(part 1 of 2)
# Autodesk Inventor assembly: eMachineShop.20
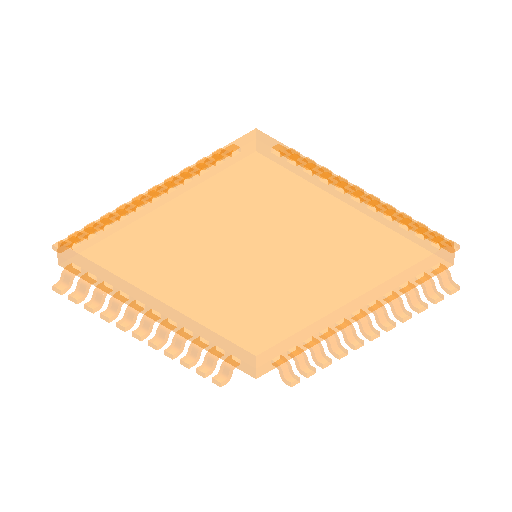
[picture p0: Inventor's stored thumbnail of the model, 512x512]
Saved by Autodesk Inventor 2026.1 (Build 301233000, 233)
## iProperties
Created: 2025-10-01
Part Number: eMachineShop.20
Document SubType Name: Assembly
Designer: gianm
Author: gianm
## Documents named in this file (583)
- D:\Tesis\Modelo 3D\CAD\Electronicos\MC15A_V5\MC15A_V5_1779569544.214\MC15A_V5_1779569544.214\eMachineShop.20.iam
- D:\Tesis\Modelo 3D\CAD\Electronicos\MC15A_V5\MC15A_V5_1779569544.214\MC15A_V5_1779569544.214\eMachineShop.20.1.ipt
- D:\Tesis\Modelo 3D\CAD\Electronicos\MC15A_V5\MC15A_V5_1779569544.214\MC15A_V5_1779569544.214\eMachineShop.20.2.ipt
- D:\Tesis\Modelo 3D\CAD\Electronicos\MC15A_V5\MC15A_V5_1779569544.214\MC15A_V5_1779569544.214\eMachineShop.20.3.ipt
- D:\Tesis\Modelo 3D\CAD\Electronicos\MC15A_V5\MC15A_V5_1779569544.214\MC15A_V5_1779569544.214\eMachineShop.20.4.ipt
- D:\Tesis\Modelo 3D\CAD\Electronicos\MC15A_V5\MC15A_V5_1779569544.214\MC15A_V5_1779569544.214\eMachineShop.20.5.ipt
- D:\Tesis\Modelo 3D\CAD\Electronicos\MC15A_V5\MC15A_V5_1779569544.214\MC15A_V5_1779569544.214\eMachineShop.20.6.ipt
- D:\Tesis\Modelo 3D\CAD\Electronicos\MC15A_V5\MC15A_V5_1779569544.214\MC15A_V5_1779569544.214\eMachineShop.20.7.ipt
- D:\Tesis\Modelo 3D\CAD\Electronicos\MC15A_V5\MC15A_V5_1779569544.214\MC15A_V5_1779569544.214\eMachineShop.20.8.ipt
- D:\Tesis\Modelo 3D\CAD\Electronicos\MC15A_V5\MC15A_V5_1779569544.214\MC15A_V5_1779569544.214\eMachineShop.20.9.ipt
- D:\Tesis\Modelo 3D\CAD\Electronicos\MC15A_V5\MC15A_V5_1779569544.214\MC15A_V5_1779569544.214\eMachineShop.20.10.ipt
- D:\Tesis\Modelo 3D\CAD\Electronicos\MC15A_V5\MC15A_V5_1779569544.214\MC15A_V5_1779569544.214\eMachineShop.20.11.ipt
- D:\Tesis\Modelo 3D\CAD\Electronicos\MC15A_V5\MC15A_V5_1779569544.214\MC15A_V5_1779569544.214\eMachineShop.20.12.ipt
- D:\Tesis\Modelo 3D\CAD\Electronicos\MC15A_V5\MC15A_V5_1779569544.214\MC15A_V5_1779569544.214\eMachineShop.20.13.ipt
- D:\Tesis\Modelo 3D\CAD\Electronicos\MC15A_V5\MC15A_V5_1779569544.214\MC15A_V5_1779569544.214\eMachineShop.20.14.ipt
- D:\Tesis\Modelo 3D\CAD\Electronicos\MC15A_V5\MC15A_V5_1779569544.214\MC15A_V5_1779569544.214\eMachineShop.20.15.ipt
- D:\Tesis\Modelo 3D\CAD\Electronicos\MC15A_V5\MC15A_V5_1779569544.214\MC15A_V5_1779569544.214\eMachineShop.20.16.ipt
- D:\Tesis\Modelo 3D\CAD\Electronicos\MC15A_V5\MC15A_V5_1779569544.214\MC15A_V5_1779569544.214\eMachineShop.20.17.ipt
- D:\Tesis\Modelo 3D\CAD\Electronicos\MC15A_V5\MC15A_V5_1779569544.214\MC15A_V5_1779569544.214\eMachineShop.20.18.ipt
- D:\Tesis\Modelo 3D\CAD\Electronicos\MC15A_V5\MC15A_V5_1779569544.214\MC15A_V5_1779569544.214\eMachineShop.20.19.ipt
- D:\Tesis\Modelo 3D\CAD\Electronicos\MC15A_V5\MC15A_V5_1779569544.214\MC15A_V5_1779569544.214\eMachineShop.20.20.ipt
- D:\Tesis\Modelo 3D\CAD\Electronicos\MC15A_V5\MC15A_V5_1779569544.214\MC15A_V5_1779569544.214\eMachineShop.20.21.ipt
- D:\Tesis\Modelo 3D\CAD\Electronicos\MC15A_V5\MC15A_V5_1779569544.214\MC15A_V5_1779569544.214\eMachineShop.20.22.ipt
- D:\Tesis\Modelo 3D\CAD\Electronicos\MC15A_V5\MC15A_V5_1779569544.214\MC15A_V5_1779569544.214\eMachineShop.20.23.ipt
- D:\Tesis\Modelo 3D\CAD\Electronicos\MC15A_V5\MC15A_V5_1779569544.214\MC15A_V5_1779569544.214\eMachineShop.20.24.ipt
- D:\Tesis\Modelo 3D\CAD\Electronicos\MC15A_V5\MC15A_V5_1779569544.214\MC15A_V5_1779569544.214\eMachineShop.20.25.ipt
- D:\Tesis\Modelo 3D\CAD\Electronicos\MC15A_V5\MC15A_V5_1779569544.214\MC15A_V5_1779569544.214\eMachineShop.20.26.ipt
- D:\Tesis\Modelo 3D\CAD\Electronicos\MC15A_V5\MC15A_V5_1779569544.214\MC15A_V5_1779569544.214\eMachineShop.20.27.ipt
- D:\Tesis\Modelo 3D\CAD\Electronicos\MC15A_V5\MC15A_V5_1779569544.214\MC15A_V5_1779569544.214\eMachineShop.20.28.ipt
- D:\Tesis\Modelo 3D\CAD\Electronicos\MC15A_V5\MC15A_V5_1779569544.214\MC15A_V5_1779569544.214\eMachineShop.20.29.ipt
- D:\Tesis\Modelo 3D\CAD\Electronicos\MC15A_V5\MC15A_V5_1779569544.214\MC15A_V5_1779569544.214\eMachineShop.20.30.ipt
- D:\Tesis\Modelo 3D\CAD\Electronicos\MC15A_V5\MC15A_V5_1779569544.214\MC15A_V5_1779569544.214\eMachineShop.20.31.ipt
- D:\Tesis\Modelo 3D\CAD\Electronicos\MC15A_V5\MC15A_V5_1779569544.214\MC15A_V5_1779569544.214\eMachineShop.20.32.ipt
- D:\Tesis\Modelo 3D\CAD\Electronicos\MC15A_V5\MC15A_V5_1779569544.214\MC15A_V5_1779569544.214\eMachineShop.20.33.ipt
- D:\Tesis\Modelo 3D\CAD\Electronicos\MC15A_V5\MC15A_V5_1779569544.214\MC15A_V5_1779569544.214\eMachineShop.20.34.ipt
- D:\Tesis\Modelo 3D\CAD\Electronicos\MC15A_V5\MC15A_V5_1779569544.214\MC15A_V5_1779569544.214\eMachineShop.20.35.ipt
- D:\Tesis\Modelo 3D\CAD\Electronicos\MC15A_V5\MC15A_V5_1779569544.214\MC15A_V5_1779569544.214\eMachineShop.20.36.ipt
- D:\Tesis\Modelo 3D\CAD\Electronicos\MC15A_V5\MC15A_V5_1779569544.214\MC15A_V5_1779569544.214\eMachineShop.20.37.ipt
- D:\Tesis\Modelo 3D\CAD\Electronicos\MC15A_V5\MC15A_V5_1779569544.214\MC15A_V5_1779569544.214\eMachineShop.20.38.ipt
- D:\Tesis\Modelo 3D\CAD\Electronicos\MC15A_V5\MC15A_V5_1779569544.214\MC15A_V5_1779569544.214\eMachineShop.20.39.ipt
- D:\Tesis\Modelo 3D\CAD\Electronicos\MC15A_V5\MC15A_V5_1779569544.214\MC15A_V5_1779569544.214\eMachineShop.20.40.ipt
- D:\Tesis\Modelo 3D\CAD\Electronicos\MC15A_V5\MC15A_V5_1779569544.214\MC15A_V5_1779569544.214\eMachineShop.20.41.ipt
- D:\Tesis\Modelo 3D\CAD\Electronicos\MC15A_V5\MC15A_V5_1779569544.214\MC15A_V5_1779569544.214\eMachineShop.20.42.ipt
- D:\Tesis\Modelo 3D\CAD\Electronicos\MC15A_V5\MC15A_V5_1779569544.214\MC15A_V5_1779569544.214\eMachineShop.20.43.ipt
- D:\Tesis\Modelo 3D\CAD\Electronicos\MC15A_V5\MC15A_V5_1779569544.214\MC15A_V5_1779569544.214\eMachineShop.20.44.ipt
- D:\Tesis\Modelo 3D\CAD\Electronicos\MC15A_V5\MC15A_V5_1779569544.214\MC15A_V5_1779569544.214\eMachineShop.20.45.ipt
- D:\Tesis\Modelo 3D\CAD\Electronicos\MC15A_V5\MC15A_V5_1779569544.214\MC15A_V5_1779569544.214\eMachineShop.20.46.ipt
- D:\Tesis\Modelo 3D\CAD\Electronicos\MC15A_V5\MC15A_V5_1779569544.214\MC15A_V5_1779569544.214\eMachineShop.20.47.ipt
- D:\Tesis\Modelo 3D\CAD\Electronicos\MC15A_V5\MC15A_V5_1779569544.214\MC15A_V5_1779569544.214\eMachineShop.20.48.ipt
- D:\Tesis\Modelo 3D\CAD\Electronicos\MC15A_V5\MC15A_V5_1779569544.214\MC15A_V5_1779569544.214\eMachineShop.20.49.ipt
- D:\Tesis\Modelo 3D\CAD\Electronicos\MC15A_V5\MC15A_V5_1779569544.214\MC15A_V5_1779569544.214\eMachineShop.20.50.ipt
- D:\Tesis\Modelo 3D\CAD\Electronicos\MC15A_V5\MC15A_V5_1779569544.214\MC15A_V5_1779569544.214\eMachineShop.20.51.ipt
- D:\Tesis\Modelo 3D\CAD\Electronicos\MC15A_V5\MC15A_V5_1779569544.214\MC15A_V5_1779569544.214\eMachineShop.20.52.ipt
- D:\Tesis\Modelo 3D\CAD\Electronicos\MC15A_V5\MC15A_V5_1779569544.214\MC15A_V5_1779569544.214\eMachineShop.20.53.ipt
- D:\Tesis\Modelo 3D\CAD\Electronicos\MC15A_V5\MC15A_V5_1779569544.214\MC15A_V5_1779569544.214\eMachineShop.20.54.ipt
- D:\Tesis\Modelo 3D\CAD\Electronicos\MC15A_V5\MC15A_V5_1779569544.214\MC15A_V5_1779569544.214\eMachineShop.20.55.ipt
- D:\Tesis\Modelo 3D\CAD\Electronicos\MC15A_V5\MC15A_V5_1779569544.214\MC15A_V5_1779569544.214\eMachineShop.20.56.ipt
- D:\Tesis\Modelo 3D\CAD\Electronicos\MC15A_V5\MC15A_V5_1779569544.214\MC15A_V5_1779569544.214\eMachineShop.20.57.ipt
- D:\Tesis\Modelo 3D\CAD\Electronicos\MC15A_V5\MC15A_V5_1779569544.214\MC15A_V5_1779569544.214\eMachineShop.20.58.ipt
- D:\Tesis\Modelo 3D\CAD\Electronicos\MC15A_V5\MC15A_V5_1779569544.214\MC15A_V5_1779569544.214\eMachineShop.20.59.ipt
- D:\Tesis\Modelo 3D\CAD\Electronicos\MC15A_V5\MC15A_V5_1779569544.214\MC15A_V5_1779569544.214\eMachineShop.20.60.ipt
- D:\Tesis\Modelo 3D\CAD\Electronicos\MC15A_V5\MC15A_V5_1779569544.214\MC15A_V5_1779569544.214\eMachineShop.20.61.ipt
- D:\Tesis\Modelo 3D\CAD\Electronicos\MC15A_V5\MC15A_V5_1779569544.214\MC15A_V5_1779569544.214\eMachineShop.20.62.ipt
- D:\Tesis\Modelo 3D\CAD\Electronicos\MC15A_V5\MC15A_V5_1779569544.214\MC15A_V5_1779569544.214\eMachineShop.20.63.ipt
- D:\Tesis\Modelo 3D\CAD\Electronicos\MC15A_V5\MC15A_V5_1779569544.214\MC15A_V5_1779569544.214\eMachineShop.20.64.ipt
- D:\Tesis\Modelo 3D\CAD\Electronicos\MC15A_V5\MC15A_V5_1779569544.214\MC15A_V5_1779569544.214\eMachineShop.20.65.ipt
- D:\Tesis\Modelo 3D\CAD\Electronicos\MC15A_V5\MC15A_V5_1779569544.214\MC15A_V5_1779569544.214\eMachineShop.20.66.ipt
- D:\Tesis\Modelo 3D\CAD\Electronicos\MC15A_V5\MC15A_V5_1779569544.214\MC15A_V5_1779569544.214\eMachineShop.20.67.ipt
- D:\Tesis\Modelo 3D\CAD\Electronicos\MC15A_V5\MC15A_V5_1779569544.214\MC15A_V5_1779569544.214\eMachineShop.20.68.ipt
- D:\Tesis\Modelo 3D\CAD\Electronicos\MC15A_V5\MC15A_V5_1779569544.214\MC15A_V5_1779569544.214\eMachineShop.20.69.ipt
- D:\Tesis\Modelo 3D\CAD\Electronicos\MC15A_V5\MC15A_V5_1779569544.214\MC15A_V5_1779569544.214\eMachineShop.20.70.ipt
- D:\Tesis\Modelo 3D\CAD\Electronicos\MC15A_V5\MC15A_V5_1779569544.214\MC15A_V5_1779569544.214\eMachineShop.20.71.ipt
- D:\Tesis\Modelo 3D\CAD\Electronicos\MC15A_V5\MC15A_V5_1779569544.214\MC15A_V5_1779569544.214\eMachineShop.20.72.ipt
- D:\Tesis\Modelo 3D\CAD\Electronicos\MC15A_V5\MC15A_V5_1779569544.214\MC15A_V5_1779569544.214\eMachineShop.20.73.ipt
- D:\Tesis\Modelo 3D\CAD\Electronicos\MC15A_V5\MC15A_V5_1779569544.214\MC15A_V5_1779569544.214\eMachineShop.20.74.ipt
- D:\Tesis\Modelo 3D\CAD\Electronicos\MC15A_V5\MC15A_V5_1779569544.214\MC15A_V5_1779569544.214\eMachineShop.20.75.ipt
- D:\Tesis\Modelo 3D\CAD\Electronicos\MC15A_V5\MC15A_V5_1779569544.214\MC15A_V5_1779569544.214\eMachineShop.20.76.ipt
- D:\Tesis\Modelo 3D\CAD\Electronicos\MC15A_V5\MC15A_V5_1779569544.214\MC15A_V5_1779569544.214\eMachineShop.20.77.ipt
- D:\Tesis\Modelo 3D\CAD\Electronicos\MC15A_V5\MC15A_V5_1779569544.214\MC15A_V5_1779569544.214\eMachineShop.20.78.ipt
- D:\Tesis\Modelo 3D\CAD\Electronicos\MC15A_V5\MC15A_V5_1779569544.214\MC15A_V5_1779569544.214\eMachineShop.20.79.ipt
- D:\Tesis\Modelo 3D\CAD\Electronicos\MC15A_V5\MC15A_V5_1779569544.214\MC15A_V5_1779569544.214\eMachineShop.20.80.ipt
- D:\Tesis\Modelo 3D\CAD\Electronicos\MC15A_V5\MC15A_V5_1779569544.214\MC15A_V5_1779569544.214\eMachineShop.20.81.ipt
- D:\Tesis\Modelo 3D\CAD\Electronicos\MC15A_V5\MC15A_V5_1779569544.214\MC15A_V5_1779569544.214\eMachineShop.20.82.ipt
- D:\Tesis\Modelo 3D\CAD\Electronicos\MC15A_V5\MC15A_V5_1779569544.214\MC15A_V5_1779569544.214\eMachineShop.20.83.ipt
- D:\Tesis\Modelo 3D\CAD\Electronicos\MC15A_V5\MC15A_V5_1779569544.214\MC15A_V5_1779569544.214\eMachineShop.20.84.ipt
- D:\Tesis\Modelo 3D\CAD\Electronicos\MC15A_V5\MC15A_V5_1779569544.214\MC15A_V5_1779569544.214\eMachineShop.20.85.ipt
- D:\Tesis\Modelo 3D\CAD\Electronicos\MC15A_V5\MC15A_V5_1779569544.214\MC15A_V5_1779569544.214\eMachineShop.20.86.ipt
- D:\Tesis\Modelo 3D\CAD\Electronicos\MC15A_V5\MC15A_V5_1779569544.214\MC15A_V5_1779569544.214\eMachineShop.20.87.ipt
- D:\Tesis\Modelo 3D\CAD\Electronicos\MC15A_V5\MC15A_V5_1779569544.214\MC15A_V5_1779569544.214\eMachineShop.20.88.ipt
- D:\Tesis\Modelo 3D\CAD\Electronicos\MC15A_V5\MC15A_V5_1779569544.214\MC15A_V5_1779569544.214\eMachineShop.20.89.ipt
- D:\Tesis\Modelo 3D\CAD\Electronicos\MC15A_V5\MC15A_V5_1779569544.214\MC15A_V5_1779569544.214\eMachineShop.20.90.ipt
- D:\Tesis\Modelo 3D\CAD\Electronicos\MC15A_V5\MC15A_V5_1779569544.214\MC15A_V5_1779569544.214\eMachineShop.20.91.ipt
- D:\Tesis\Modelo 3D\CAD\Electronicos\MC15A_V5\MC15A_V5_1779569544.214\MC15A_V5_1779569544.214\eMachineShop.20.92.ipt
- D:\Tesis\Modelo 3D\CAD\Electronicos\MC15A_V5\MC15A_V5_1779569544.214\MC15A_V5_1779569544.214\eMachineShop.20.93.ipt
- D:\Tesis\Modelo 3D\CAD\Electronicos\MC15A_V5\MC15A_V5_1779569544.214\MC15A_V5_1779569544.214\eMachineShop.20.94.ipt
- D:\Tesis\Modelo 3D\CAD\Electronicos\MC15A_V5\MC15A_V5_1779569544.214\MC15A_V5_1779569544.214\eMachineShop.20.95.ipt
- D:\Tesis\Modelo 3D\CAD\Electronicos\MC15A_V5\MC15A_V5_1779569544.214\MC15A_V5_1779569544.214\eMachineShop.20.96.ipt
- D:\Tesis\Modelo 3D\CAD\Electronicos\MC15A_V5\MC15A_V5_1779569544.214\MC15A_V5_1779569544.214\eMachineShop.20.97.ipt
- D:\Tesis\Modelo 3D\CAD\Electronicos\MC15A_V5\MC15A_V5_1779569544.214\MC15A_V5_1779569544.214\eMachineShop.20.98.ipt
- D:\Tesis\Modelo 3D\CAD\Electronicos\MC15A_V5\MC15A_V5_1779569544.214\MC15A_V5_1779569544.214\eMachineShop.20.99.ipt
- D:\Tesis\Modelo 3D\CAD\Electronicos\MC15A_V5\MC15A_V5_1779569544.214\MC15A_V5_1779569544.214\eMachineShop.20.100.ipt
- D:\Tesis\Modelo 3D\CAD\Electronicos\MC15A_V5\MC15A_V5_1779569544.214\MC15A_V5_1779569544.214\eMachineShop.20.101.ipt
- D:\Tesis\Modelo 3D\CAD\Electronicos\MC15A_V5\MC15A_V5_1779569544.214\MC15A_V5_1779569544.214\eMachineShop.20.102.ipt
- D:\Tesis\Modelo 3D\CAD\Electronicos\MC15A_V5\MC15A_V5_1779569544.214\MC15A_V5_1779569544.214\eMachineShop.20.103.ipt
- D:\Tesis\Modelo 3D\CAD\Electronicos\MC15A_V5\MC15A_V5_1779569544.214\MC15A_V5_1779569544.214\eMachineShop.20.104.ipt
- D:\Tesis\Modelo 3D\CAD\Electronicos\MC15A_V5\MC15A_V5_1779569544.214\MC15A_V5_1779569544.214\eMachineShop.20.105.ipt
- D:\Tesis\Modelo 3D\CAD\Electronicos\MC15A_V5\MC15A_V5_1779569544.214\MC15A_V5_1779569544.214\eMachineShop.20.106.ipt
- D:\Tesis\Modelo 3D\CAD\Electronicos\MC15A_V5\MC15A_V5_1779569544.214\MC15A_V5_1779569544.214\eMachineShop.20.107.ipt
- D:\Tesis\Modelo 3D\CAD\Electronicos\MC15A_V5\MC15A_V5_1779569544.214\MC15A_V5_1779569544.214\eMachineShop.20.108.ipt
- D:\Tesis\Modelo 3D\CAD\Electronicos\MC15A_V5\MC15A_V5_1779569544.214\MC15A_V5_1779569544.214\eMachineShop.20.109.ipt
- D:\Tesis\Modelo 3D\CAD\Electronicos\MC15A_V5\MC15A_V5_1779569544.214\MC15A_V5_1779569544.214\eMachineShop.20.110.ipt
- D:\Tesis\Modelo 3D\CAD\Electronicos\MC15A_V5\MC15A_V5_1779569544.214\MC15A_V5_1779569544.214\eMachineShop.20.111.ipt
- D:\Tesis\Modelo 3D\CAD\Electronicos\MC15A_V5\MC15A_V5_1779569544.214\MC15A_V5_1779569544.214\eMachineShop.20.112.ipt
- D:\Tesis\Modelo 3D\CAD\Electronicos\MC15A_V5\MC15A_V5_1779569544.214\MC15A_V5_1779569544.214\eMachineShop.20.113.ipt
- D:\Tesis\Modelo 3D\CAD\Electronicos\MC15A_V5\MC15A_V5_1779569544.214\MC15A_V5_1779569544.214\eMachineShop.20.114.ipt
- D:\Tesis\Modelo 3D\CAD\Electronicos\MC15A_V5\MC15A_V5_1779569544.214\MC15A_V5_1779569544.214\eMachineShop.20.115.ipt
- D:\Tesis\Modelo 3D\CAD\Electronicos\MC15A_V5\MC15A_V5_1779569544.214\MC15A_V5_1779569544.214\eMachineShop.20.116.ipt
- D:\Tesis\Modelo 3D\CAD\Electronicos\MC15A_V5\MC15A_V5_1779569544.214\MC15A_V5_1779569544.214\eMachineShop.20.117.ipt
- D:\Tesis\Modelo 3D\CAD\Electronicos\MC15A_V5\MC15A_V5_1779569544.214\MC15A_V5_1779569544.214\eMachineShop.20.118.ipt
- D:\Tesis\Modelo 3D\CAD\Electronicos\MC15A_V5\MC15A_V5_1779569544.214\MC15A_V5_1779569544.214\eMachineShop.20.119.ipt
- D:\Tesis\Modelo 3D\CAD\Electronicos\MC15A_V5\MC15A_V5_1779569544.214\MC15A_V5_1779569544.214\eMachineShop.20.120.ipt
- D:\Tesis\Modelo 3D\CAD\Electronicos\MC15A_V5\MC15A_V5_1779569544.214\MC15A_V5_1779569544.214\eMachineShop.20.121.ipt
- D:\Tesis\Modelo 3D\CAD\Electronicos\MC15A_V5\MC15A_V5_1779569544.214\MC15A_V5_1779569544.214\eMachineShop.20.122.ipt
- D:\Tesis\Modelo 3D\CAD\Electronicos\MC15A_V5\MC15A_V5_1779569544.214\MC15A_V5_1779569544.214\eMachineShop.20.123.ipt
- D:\Tesis\Modelo 3D\CAD\Electronicos\MC15A_V5\MC15A_V5_1779569544.214\MC15A_V5_1779569544.214\eMachineShop.20.124.ipt
- D:\Tesis\Modelo 3D\CAD\Electronicos\MC15A_V5\MC15A_V5_1779569544.214\MC15A_V5_1779569544.214\eMachineShop.20.125.ipt
- D:\Tesis\Modelo 3D\CAD\Electronicos\MC15A_V5\MC15A_V5_1779569544.214\MC15A_V5_1779569544.214\eMachineShop.20.126.ipt
- D:\Tesis\Modelo 3D\CAD\Electronicos\MC15A_V5\MC15A_V5_1779569544.214\MC15A_V5_1779569544.214\eMachineShop.20.127.ipt
- D:\Tesis\Modelo 3D\CAD\Electronicos\MC15A_V5\MC15A_V5_1779569544.214\MC15A_V5_1779569544.214\eMachineShop.20.128.ipt
- D:\Tesis\Modelo 3D\CAD\Electronicos\MC15A_V5\MC15A_V5_1779569544.214\MC15A_V5_1779569544.214\eMachineShop.20.129.ipt
- D:\Tesis\Modelo 3D\CAD\Electronicos\MC15A_V5\MC15A_V5_1779569544.214\MC15A_V5_1779569544.214\eMachineShop.20.130.ipt
- D:\Tesis\Modelo 3D\CAD\Electronicos\MC15A_V5\MC15A_V5_1779569544.214\MC15A_V5_1779569544.214\eMachineShop.20.131.ipt
- D:\Tesis\Modelo 3D\CAD\Electronicos\MC15A_V5\MC15A_V5_1779569544.214\MC15A_V5_1779569544.214\eMachineShop.20.132.ipt
- D:\Tesis\Modelo 3D\CAD\Electronicos\MC15A_V5\MC15A_V5_1779569544.214\MC15A_V5_1779569544.214\eMachineShop.20.133.ipt
- D:\Tesis\Modelo 3D\CAD\Electronicos\MC15A_V5\MC15A_V5_1779569544.214\MC15A_V5_1779569544.214\eMachineShop.20.134.ipt
- D:\Tesis\Modelo 3D\CAD\Electronicos\MC15A_V5\MC15A_V5_1779569544.214\MC15A_V5_1779569544.214\eMachineShop.20.135.ipt
- D:\Tesis\Modelo 3D\CAD\Electronicos\MC15A_V5\MC15A_V5_1779569544.214\MC15A_V5_1779569544.214\eMachineShop.20.136.ipt
- D:\Tesis\Modelo 3D\CAD\Electronicos\MC15A_V5\MC15A_V5_1779569544.214\MC15A_V5_1779569544.214\eMachineShop.20.137.ipt
- D:\Tesis\Modelo 3D\CAD\Electronicos\MC15A_V5\MC15A_V5_1779569544.214\MC15A_V5_1779569544.214\eMachineShop.20.138.ipt
- D:\Tesis\Modelo 3D\CAD\Electronicos\MC15A_V5\MC15A_V5_1779569544.214\MC15A_V5_1779569544.214\eMachineShop.20.139.ipt
- D:\Tesis\Modelo 3D\CAD\Electronicos\MC15A_V5\MC15A_V5_1779569544.214\MC15A_V5_1779569544.214\eMachineShop.20.140.ipt
- D:\Tesis\Modelo 3D\CAD\Electronicos\MC15A_V5\MC15A_V5_1779569544.214\MC15A_V5_1779569544.214\eMachineShop.20.141.ipt
- D:\Tesis\Modelo 3D\CAD\Electronicos\MC15A_V5\MC15A_V5_1779569544.214\MC15A_V5_1779569544.214\eMachineShop.20.142.ipt
- D:\Tesis\Modelo 3D\CAD\Electronicos\MC15A_V5\MC15A_V5_1779569544.214\MC15A_V5_1779569544.214\eMachineShop.20.143.ipt
- D:\Tesis\Modelo 3D\CAD\Electronicos\MC15A_V5\MC15A_V5_1779569544.214\MC15A_V5_1779569544.214\eMachineShop.20.144.ipt
- D:\Tesis\Modelo 3D\CAD\Electronicos\MC15A_V5\MC15A_V5_1779569544.214\MC15A_V5_1779569544.214\eMachineShop.20.145.ipt
- D:\Tesis\Modelo 3D\CAD\Electronicos\MC15A_V5\MC15A_V5_1779569544.214\MC15A_V5_1779569544.214\eMachineShop.20.146.ipt
- D:\Tesis\Modelo 3D\CAD\Electronicos\MC15A_V5\MC15A_V5_1779569544.214\MC15A_V5_1779569544.214\eMachineShop.20.147.ipt
- D:\Tesis\Modelo 3D\CAD\Electronicos\MC15A_V5\MC15A_V5_1779569544.214\MC15A_V5_1779569544.214\eMachineShop.20.148.ipt
- D:\Tesis\Modelo 3D\CAD\Electronicos\MC15A_V5\MC15A_V5_1779569544.214\MC15A_V5_1779569544.214\eMachineShop.20.149.ipt
- D:\Tesis\Modelo 3D\CAD\Electronicos\MC15A_V5\MC15A_V5_1779569544.214\MC15A_V5_1779569544.214\eMachineShop.20.150.ipt
- D:\Tesis\Modelo 3D\CAD\Electronicos\MC15A_V5\MC15A_V5_1779569544.214\MC15A_V5_1779569544.214\eMachineShop.20.151.ipt
- D:\Tesis\Modelo 3D\CAD\Electronicos\MC15A_V5\MC15A_V5_1779569544.214\MC15A_V5_1779569544.214\eMachineShop.20.152.ipt
- D:\Tesis\Modelo 3D\CAD\Electronicos\MC15A_V5\MC15A_V5_1779569544.214\MC15A_V5_1779569544.214\eMachineShop.20.153.ipt
- D:\Tesis\Modelo 3D\CAD\Electronicos\MC15A_V5\MC15A_V5_1779569544.214\MC15A_V5_1779569544.214\eMachineShop.20.154.ipt
- D:\Tesis\Modelo 3D\CAD\Electronicos\MC15A_V5\MC15A_V5_1779569544.214\MC15A_V5_1779569544.214\eMachineShop.20.155.ipt
- D:\Tesis\Modelo 3D\CAD\Electronicos\MC15A_V5\MC15A_V5_1779569544.214\MC15A_V5_1779569544.214\eMachineShop.20.156.ipt
- D:\Tesis\Modelo 3D\CAD\Electronicos\MC15A_V5\MC15A_V5_1779569544.214\MC15A_V5_1779569544.214\eMachineShop.20.157.ipt
- D:\Tesis\Modelo 3D\CAD\Electronicos\MC15A_V5\MC15A_V5_1779569544.214\MC15A_V5_1779569544.214\eMachineShop.20.158.ipt
- D:\Tesis\Modelo 3D\CAD\Electronicos\MC15A_V5\MC15A_V5_1779569544.214\MC15A_V5_1779569544.214\eMachineShop.20.159.ipt
- D:\Tesis\Modelo 3D\CAD\Electronicos\MC15A_V5\MC15A_V5_1779569544.214\MC15A_V5_1779569544.214\eMachineShop.20.160.ipt
- D:\Tesis\Modelo 3D\CAD\Electronicos\MC15A_V5\MC15A_V5_1779569544.214\MC15A_V5_1779569544.214\eMachineShop.20.161.ipt
- D:\Tesis\Modelo 3D\CAD\Electronicos\MC15A_V5\MC15A_V5_1779569544.214\MC15A_V5_1779569544.214\eMachineShop.20.162.ipt
- D:\Tesis\Modelo 3D\CAD\Electronicos\MC15A_V5\MC15A_V5_1779569544.214\MC15A_V5_1779569544.214\eMachineShop.20.163.ipt
- D:\Tesis\Modelo 3D\CAD\Electronicos\MC15A_V5\MC15A_V5_1779569544.214\MC15A_V5_1779569544.214\eMachineShop.20.164.ipt
- D:\Tesis\Modelo 3D\CAD\Electronicos\MC15A_V5\MC15A_V5_1779569544.214\MC15A_V5_1779569544.214\eMachineShop.20.165.ipt
- D:\Tesis\Modelo 3D\CAD\Electronicos\MC15A_V5\MC15A_V5_1779569544.214\MC15A_V5_1779569544.214\eMachineShop.20.166.ipt
- D:\Tesis\Modelo 3D\CAD\Electronicos\MC15A_V5\MC15A_V5_1779569544.214\MC15A_V5_1779569544.214\eMachineShop.20.167.ipt
- D:\Tesis\Modelo 3D\CAD\Electronicos\MC15A_V5\MC15A_V5_1779569544.214\MC15A_V5_1779569544.214\eMachineShop.20.168.ipt
- D:\Tesis\Modelo 3D\CAD\Electronicos\MC15A_V5\MC15A_V5_1779569544.214\MC15A_V5_1779569544.214\eMachineShop.20.169.ipt
- D:\Tesis\Modelo 3D\CAD\Electronicos\MC15A_V5\MC15A_V5_1779569544.214\MC15A_V5_1779569544.214\eMachineShop.20.170.ipt
- D:\Tesis\Modelo 3D\CAD\Electronicos\MC15A_V5\MC15A_V5_1779569544.214\MC15A_V5_1779569544.214\eMachineShop.20.171.ipt
- D:\Tesis\Modelo 3D\CAD\Electronicos\MC15A_V5\MC15A_V5_1779569544.214\MC15A_V5_1779569544.214\eMachineShop.20.172.ipt
- D:\Tesis\Modelo 3D\CAD\Electronicos\MC15A_V5\MC15A_V5_1779569544.214\MC15A_V5_1779569544.214\eMachineShop.20.173.ipt
- D:\Tesis\Modelo 3D\CAD\Electronicos\MC15A_V5\MC15A_V5_1779569544.214\MC15A_V5_1779569544.214\eMachineShop.20.174.ipt
- D:\Tesis\Modelo 3D\CAD\Electronicos\MC15A_V5\MC15A_V5_1779569544.214\MC15A_V5_1779569544.214\eMachineShop.20.175.ipt
- D:\Tesis\Modelo 3D\CAD\Electronicos\MC15A_V5\MC15A_V5_1779569544.214\MC15A_V5_1779569544.214\eMachineShop.20.176.ipt
- D:\Tesis\Modelo 3D\CAD\Electronicos\MC15A_V5\MC15A_V5_1779569544.214\MC15A_V5_1779569544.214\eMachineShop.20.177.ipt
- D:\Tesis\Modelo 3D\CAD\Electronicos\MC15A_V5\MC15A_V5_1779569544.214\MC15A_V5_1779569544.214\eMachineShop.20.178.ipt
- D:\Tesis\Modelo 3D\CAD\Electronicos\MC15A_V5\MC15A_V5_1779569544.214\MC15A_V5_1779569544.214\eMachineShop.20.179.ipt
- D:\Tesis\Modelo 3D\CAD\Electronicos\MC15A_V5\MC15A_V5_1779569544.214\MC15A_V5_1779569544.214\eMachineShop.20.180.ipt
- D:\Tesis\Modelo 3D\CAD\Electronicos\MC15A_V5\MC15A_V5_1779569544.214\MC15A_V5_1779569544.214\eMachineShop.20.181.ipt
- D:\Tesis\Modelo 3D\CAD\Electronicos\MC15A_V5\MC15A_V5_1779569544.214\MC15A_V5_1779569544.214\eMachineShop.20.182.ipt
- D:\Tesis\Modelo 3D\CAD\Electronicos\MC15A_V5\MC15A_V5_1779569544.214\MC15A_V5_1779569544.214\eMachineShop.20.183.ipt
- D:\Tesis\Modelo 3D\CAD\Electronicos\MC15A_V5\MC15A_V5_1779569544.214\MC15A_V5_1779569544.214\eMachineShop.20.184.ipt
- D:\Tesis\Modelo 3D\CAD\Electronicos\MC15A_V5\MC15A_V5_1779569544.214\MC15A_V5_1779569544.214\eMachineShop.20.185.ipt
- D:\Tesis\Modelo 3D\CAD\Electronicos\MC15A_V5\MC15A_V5_1779569544.214\MC15A_V5_1779569544.214\eMachineShop.20.186.ipt
- D:\Tesis\Modelo 3D\CAD\Electronicos\MC15A_V5\MC15A_V5_1779569544.214\MC15A_V5_1779569544.214\eMachineShop.20.187.ipt
- D:\Tesis\Modelo 3D\CAD\Electronicos\MC15A_V5\MC15A_V5_1779569544.214\MC15A_V5_1779569544.214\eMachineShop.20.188.ipt
- D:\Tesis\Modelo 3D\CAD\Electronicos\MC15A_V5\MC15A_V5_1779569544.214\MC15A_V5_1779569544.214\eMachineShop.20.189.ipt
- D:\Tesis\Modelo 3D\CAD\Electronicos\MC15A_V5\MC15A_V5_1779569544.214\MC15A_V5_1779569544.214\eMachineShop.20.190.ipt
- D:\Tesis\Modelo 3D\CAD\Electronicos\MC15A_V5\MC15A_V5_1779569544.214\MC15A_V5_1779569544.214\eMachineShop.20.191.ipt
- D:\Tesis\Modelo 3D\CAD\Electronicos\MC15A_V5\MC15A_V5_1779569544.214\MC15A_V5_1779569544.214\eMachineShop.20.192.ipt
- D:\Tesis\Modelo 3D\CAD\Electronicos\MC15A_V5\MC15A_V5_1779569544.214\MC15A_V5_1779569544.214\eMachineShop.20.193.ipt
- D:\Tesis\Modelo 3D\CAD\Electronicos\MC15A_V5\MC15A_V5_1779569544.214\MC15A_V5_1779569544.214\eMachineShop.20.194.ipt
- D:\Tesis\Modelo 3D\CAD\Electronicos\MC15A_V5\MC15A_V5_1779569544.214\MC15A_V5_1779569544.214\eMachineShop.20.195.ipt
- D:\Tesis\Modelo 3D\CAD\Electronicos\MC15A_V5\MC15A_V5_1779569544.214\MC15A_V5_1779569544.214\eMachineShop.20.196.ipt
- D:\Tesis\Modelo 3D\CAD\Electronicos\MC15A_V5\MC15A_V5_1779569544.214\MC15A_V5_1779569544.214\eMachineShop.20.197.ipt
- D:\Tesis\Modelo 3D\CAD\Electronicos\MC15A_V5\MC15A_V5_1779569544.214\MC15A_V5_1779569544.214\eMachineShop.20.198.ipt
- D:\Tesis\Modelo 3D\CAD\Electronicos\MC15A_V5\MC15A_V5_1779569544.214\MC15A_V5_1779569544.214\eMachineShop.20.199.ipt
- D:\Tesis\Modelo 3D\CAD\Electronicos\MC15A_V5\MC15A_V5_1779569544.214\MC15A_V5_1779569544.214\eMachineShop.20.200.ipt
- D:\Tesis\Modelo 3D\CAD\Electronicos\MC15A_V5\MC15A_V5_1779569544.214\MC15A_V5_1779569544.214\eMachineShop.20.201.ipt
- D:\Tesis\Modelo 3D\CAD\Electronicos\MC15A_V5\MC15A_V5_1779569544.214\MC15A_V5_1779569544.214\eMachineShop.20.202.ipt
- D:\Tesis\Modelo 3D\CAD\Electronicos\MC15A_V5\MC15A_V5_1779569544.214\MC15A_V5_1779569544.214\eMachineShop.20.203.ipt
- D:\Tesis\Modelo 3D\CAD\Electronicos\MC15A_V5\MC15A_V5_1779569544.214\MC15A_V5_1779569544.214\eMachineShop.20.204.ipt
- D:\Tesis\Modelo 3D\CAD\Electronicos\MC15A_V5\MC15A_V5_1779569544.214\MC15A_V5_1779569544.214\eMachineShop.20.205.ipt
- D:\Tesis\Modelo 3D\CAD\Electronicos\MC15A_V5\MC15A_V5_1779569544.214\MC15A_V5_1779569544.214\eMachineShop.20.206.ipt
- D:\Tesis\Modelo 3D\CAD\Electronicos\MC15A_V5\MC15A_V5_1779569544.214\MC15A_V5_1779569544.214\eMachineShop.20.207.ipt
- D:\Tesis\Modelo 3D\CAD\Electronicos\MC15A_V5\MC15A_V5_1779569544.214\MC15A_V5_1779569544.214\eMachineShop.20.208.ipt
- D:\Tesis\Modelo 3D\CAD\Electronicos\MC15A_V5\MC15A_V5_1779569544.214\MC15A_V5_1779569544.214\eMachineShop.20.209.ipt
- D:\Tesis\Modelo 3D\CAD\Electronicos\MC15A_V5\MC15A_V5_1779569544.214\MC15A_V5_1779569544.214\eMachineShop.20.210.ipt
- D:\Tesis\Modelo 3D\CAD\Electronicos\MC15A_V5\MC15A_V5_1779569544.214\MC15A_V5_1779569544.214\eMachineShop.20.211.ipt
- D:\Tesis\Modelo 3D\CAD\Electronicos\MC15A_V5\MC15A_V5_1779569544.214\MC15A_V5_1779569544.214\eMachineShop.20.212.ipt
- D:\Tesis\Modelo 3D\CAD\Electronicos\MC15A_V5\MC15A_V5_1779569544.214\MC15A_V5_1779569544.214\eMachineShop.20.213.ipt
- D:\Tesis\Modelo 3D\CAD\Electronicos\MC15A_V5\MC15A_V5_1779569544.214\MC15A_V5_1779569544.214\eMachineShop.20.214.ipt
- D:\Tesis\Modelo 3D\CAD\Electronicos\MC15A_V5\MC15A_V5_1779569544.214\MC15A_V5_1779569544.214\eMachineShop.20.215.ipt
- D:\Tesis\Modelo 3D\CAD\Electronicos\MC15A_V5\MC15A_V5_1779569544.214\MC15A_V5_1779569544.214\eMachineShop.20.216.ipt
- D:\Tesis\Modelo 3D\CAD\Electronicos\MC15A_V5\MC15A_V5_1779569544.214\MC15A_V5_1779569544.214\eMachineShop.20.217.ipt
- D:\Tesis\Modelo 3D\CAD\Electronicos\MC15A_V5\MC15A_V5_1779569544.214\MC15A_V5_1779569544.214\eMachineShop.20.218.ipt
- D:\Tesis\Modelo 3D\CAD\Electronicos\MC15A_V5\MC15A_V5_1779569544.214\MC15A_V5_1779569544.214\eMachineShop.20.219.ipt
- D:\Tesis\Modelo 3D\CAD\Electronicos\MC15A_V5\MC15A_V5_1779569544.214\MC15A_V5_1779569544.214\eMachineShop.20.220.ipt
- D:\Tesis\Modelo 3D\CAD\Electronicos\MC15A_V5\MC15A_V5_1779569544.214\MC15A_V5_1779569544.214\eMachineShop.20.221.ipt
- D:\Tesis\Modelo 3D\CAD\Electronicos\MC15A_V5\MC15A_V5_1779569544.214\MC15A_V5_1779569544.214\eMachineShop.20.222.ipt
- D:\Tesis\Modelo 3D\CAD\Electronicos\MC15A_V5\MC15A_V5_1779569544.214\MC15A_V5_1779569544.214\eMachineShop.20.223.ipt
- D:\Tesis\Modelo 3D\CAD\Electronicos\MC15A_V5\MC15A_V5_1779569544.214\MC15A_V5_1779569544.214\eMachineShop.20.224.ipt
- D:\Tesis\Modelo 3D\CAD\Electronicos\MC15A_V5\MC15A_V5_1779569544.214\MC15A_V5_1779569544.214\eMachineShop.20.225.ipt
- D:\Tesis\Modelo 3D\CAD\Electronicos\MC15A_V5\MC15A_V5_1779569544.214\MC15A_V5_1779569544.214\eMachineShop.20.226.ipt
- D:\Tesis\Modelo 3D\CAD\Electronicos\MC15A_V5\MC15A_V5_1779569544.214\MC15A_V5_1779569544.214\eMachineShop.20.227.ipt
- D:\Tesis\Modelo 3D\CAD\Electronicos\MC15A_V5\MC15A_V5_1779569544.214\MC15A_V5_1779569544.214\eMachineShop.20.228.ipt
- D:\Tesis\Modelo 3D\CAD\Electronicos\MC15A_V5\MC15A_V5_1779569544.214\MC15A_V5_1779569544.214\eMachineShop.20.229.ipt
- D:\Tesis\Modelo 3D\CAD\Electronicos\MC15A_V5\MC15A_V5_1779569544.214\MC15A_V5_1779569544.214\eMachineShop.20.230.ipt
- D:\Tesis\Modelo 3D\CAD\Electronicos\MC15A_V5\MC15A_V5_1779569544.214\MC15A_V5_1779569544.214\eMachineShop.20.231.ipt
- D:\Tesis\Modelo 3D\CAD\Electronicos\MC15A_V5\MC15A_V5_1779569544.214\MC15A_V5_1779569544.214\eMachineShop.20.232.ipt
- D:\Tesis\Modelo 3D\CAD\Electronicos\MC15A_V5\MC15A_V5_1779569544.214\MC15A_V5_1779569544.214\eMachineShop.20.233.ipt
- D:\Tesis\Modelo 3D\CAD\Electronicos\MC15A_V5\MC15A_V5_1779569544.214\MC15A_V5_1779569544.214\eMachineShop.20.234.ipt
- D:\Tesis\Modelo 3D\CAD\Electronicos\MC15A_V5\MC15A_V5_1779569544.214\MC15A_V5_1779569544.214\eMachineShop.20.235.ipt
- D:\Tesis\Modelo 3D\CAD\Electronicos\MC15A_V5\MC15A_V5_1779569544.214\MC15A_V5_1779569544.214\eMachineShop.20.236.ipt
- D:\Tesis\Modelo 3D\CAD\Electronicos\MC15A_V5\MC15A_V5_1779569544.214\MC15A_V5_1779569544.214\eMachineShop.20.237.ipt
- D:\Tesis\Modelo 3D\CAD\Electronicos\MC15A_V5\MC15A_V5_1779569544.214\MC15A_V5_1779569544.214\eMachineShop.20.238.ipt
- D:\Tesis\Modelo 3D\CAD\Electronicos\MC15A_V5\MC15A_V5_1779569544.214\MC15A_V5_1779569544.214\eMachineShop.20.239.ipt
- D:\Tesis\Modelo 3D\CAD\Electronicos\MC15A_V5\MC15A_V5_1779569544.214\MC15A_V5_1779569544.214\eMachineShop.20.240.ipt
- D:\Tesis\Modelo 3D\CAD\Electronicos\MC15A_V5\MC15A_V5_1779569544.214\MC15A_V5_1779569544.214\eMachineShop.20.241.ipt
- D:\Tesis\Modelo 3D\CAD\Electronicos\MC15A_V5\MC15A_V5_1779569544.214\MC15A_V5_1779569544.214\eMachineShop.20.242.ipt
- D:\Tesis\Modelo 3D\CAD\Electronicos\MC15A_V5\MC15A_V5_1779569544.214\MC15A_V5_1779569544.214\eMachineShop.20.243.ipt
- D:\Tesis\Modelo 3D\CAD\Electronicos\MC15A_V5\MC15A_V5_1779569544.214\MC15A_V5_1779569544.214\eMachineShop.20.244.ipt
- D:\Tesis\Modelo 3D\CAD\Electronicos\MC15A_V5\MC15A_V5_1779569544.214\MC15A_V5_1779569544.214\eMachineShop.20.245.ipt
- D:\Tesis\Modelo 3D\CAD\Electronicos\MC15A_V5\MC15A_V5_1779569544.214\MC15A_V5_1779569544.214\eMachineShop.20.246.ipt
- D:\Tesis\Modelo 3D\CAD\Electronicos\MC15A_V5\MC15A_V5_1779569544.214\MC15A_V5_1779569544.214\eMachineShop.20.247.ipt
- D:\Tesis\Modelo 3D\CAD\Electronicos\MC15A_V5\MC15A_V5_1779569544.214\MC15A_V5_1779569544.214\eMachineShop.20.248.ipt
- D:\Tesis\Modelo 3D\CAD\Electronicos\MC15A_V5\MC15A_V5_1779569544.214\MC15A_V5_1779569544.214\eMachineShop.20.249.ipt
- D:\Tesis\Modelo 3D\CAD\Electronicos\MC15A_V5\MC15A_V5_1779569544.214\MC15A_V5_1779569544.214\eMachineShop.20.250.ipt
- D:\Tesis\Modelo 3D\CAD\Electronicos\MC15A_V5\MC15A_V5_1779569544.214\MC15A_V5_1779569544.214\eMachineShop.20.251.ipt
- D:\Tesis\Modelo 3D\CAD\Electronicos\MC15A_V5\MC15A_V5_1779569544.214\MC15A_V5_1779569544.214\eMachineShop.20.252.ipt
- D:\Tesis\Modelo 3D\CAD\Electronicos\MC15A_V5\MC15A_V5_1779569544.214\MC15A_V5_1779569544.214\eMachineShop.20.253.ipt
- D:\Tesis\Modelo 3D\CAD\Electronicos\MC15A_V5\MC15A_V5_1779569544.214\MC15A_V5_1779569544.214\eMachineShop.20.254.ipt
- D:\Tesis\Modelo 3D\CAD\Electronicos\MC15A_V5\MC15A_V5_1779569544.214\MC15A_V5_1779569544.214\eMachineShop.20.255.ipt
- D:\Tesis\Modelo 3D\CAD\Electronicos\MC15A_V5\MC15A_V5_1779569544.214\MC15A_V5_1779569544.214\eMachineShop.20.256.ipt
- D:\Tesis\Modelo 3D\CAD\Electronicos\MC15A_V5\MC15A_V5_1779569544.214\MC15A_V5_1779569544.214\eMachineShop.20.257.ipt
- D:\Tesis\Modelo 3D\CAD\Electronicos\MC15A_V5\MC15A_V5_1779569544.214\MC15A_V5_1779569544.214\eMachineShop.20.258.ipt
- D:\Tesis\Modelo 3D\CAD\Electronicos\MC15A_V5\MC15A_V5_1779569544.214\MC15A_V5_1779569544.214\eMachineShop.20.259.ipt
- D:\Tesis\Modelo 3D\CAD\Electronicos\MC15A_V5\MC15A_V5_1779569544.214\MC15A_V5_1779569544.214\eMachineShop.20.260.ipt
- D:\Tesis\Modelo 3D\CAD\Electronicos\MC15A_V5\MC15A_V5_1779569544.214\MC15A_V5_1779569544.214\eMachineShop.20.261.ipt
- D:\Tesis\Modelo 3D\CAD\Electronicos\MC15A_V5\MC15A_V5_1779569544.214\MC15A_V5_1779569544.214\eMachineShop.20.262.ipt
- D:\Tesis\Modelo 3D\CAD\Electronicos\MC15A_V5\MC15A_V5_1779569544.214\MC15A_V5_1779569544.214\eMachineShop.20.263.ipt
- D:\Tesis\Modelo 3D\CAD\Electronicos\MC15A_V5\MC15A_V5_1779569544.214\MC15A_V5_1779569544.214\eMachineShop.20.264.ipt
- D:\Tesis\Modelo 3D\CAD\Electronicos\MC15A_V5\MC15A_V5_1779569544.214\MC15A_V5_1779569544.214\eMachineShop.20.265.ipt
- D:\Tesis\Modelo 3D\CAD\Electronicos\MC15A_V5\MC15A_V5_1779569544.214\MC15A_V5_1779569544.214\eMachineShop.20.266.ipt
- D:\Tesis\Modelo 3D\CAD\Electronicos\MC15A_V5\MC15A_V5_1779569544.214\MC15A_V5_1779569544.214\eMachineShop.20.267.ipt
- D:\Tesis\Modelo 3D\CAD\Electronicos\MC15A_V5\MC15A_V5_1779569544.214\MC15A_V5_1779569544.214\eMachineShop.20.268.ipt
- D:\Tesis\Modelo 3D\CAD\Electronicos\MC15A_V5\MC15A_V5_1779569544.214\MC15A_V5_1779569544.214\eMachineShop.20.269.ipt
- D:\Tesis\Modelo 3D\CAD\Electronicos\MC15A_V5\MC15A_V5_1779569544.214\MC15A_V5_1779569544.214\eMachineShop.20.270.ipt
- D:\Tesis\Modelo 3D\CAD\Electronicos\MC15A_V5\MC15A_V5_1779569544.214\MC15A_V5_1779569544.214\eMachineShop.20.271.ipt
- D:\Tesis\Modelo 3D\CAD\Electronicos\MC15A_V5\MC15A_V5_1779569544.214\MC15A_V5_1779569544.214\eMachineShop.20.272.ipt
- D:\Tesis\Modelo 3D\CAD\Electronicos\MC15A_V5\MC15A_V5_1779569544.214\MC15A_V5_1779569544.214\eMachineShop.20.273.ipt
- D:\Tesis\Modelo 3D\CAD\Electronicos\MC15A_V5\MC15A_V5_1779569544.214\MC15A_V5_1779569544.214\eMachineShop.20.274.ipt
- D:\Tesis\Modelo 3D\CAD\Electronicos\MC15A_V5\MC15A_V5_1779569544.214\MC15A_V5_1779569544.214\eMachineShop.20.275.ipt
- D:\Tesis\Modelo 3D\CAD\Electronicos\MC15A_V5\MC15A_V5_1779569544.214\MC15A_V5_1779569544.214\eMachineShop.20.276.ipt
- D:\Tesis\Modelo 3D\CAD\Electronicos\MC15A_V5\MC15A_V5_1779569544.214\MC15A_V5_1779569544.214\eMachineShop.20.277.ipt
- D:\Tesis\Modelo 3D\CAD\Electronicos\MC15A_V5\MC15A_V5_1779569544.214\MC15A_V5_1779569544.214\eMachineShop.20.278.ipt
- D:\Tesis\Modelo 3D\CAD\Electronicos\MC15A_V5\MC15A_V5_1779569544.214\MC15A_V5_1779569544.214\eMachineShop.20.279.ipt
- D:\Tesis\Modelo 3D\CAD\Electronicos\MC15A_V5\MC15A_V5_1779569544.214\MC15A_V5_1779569544.214\eMachineShop.20.280.ipt
- D:\Tesis\Modelo 3D\CAD\Electronicos\MC15A_V5\MC15A_V5_1779569544.214\MC15A_V5_1779569544.214\eMachineShop.20.281.ipt
- D:\Tesis\Modelo 3D\CAD\Electronicos\MC15A_V5\MC15A_V5_1779569544.214\MC15A_V5_1779569544.214\eMachineShop.20.282.ipt
- D:\Tesis\Modelo 3D\CAD\Electronicos\MC15A_V5\MC15A_V5_1779569544.214\MC15A_V5_1779569544.214\eMachineShop.20.283.ipt
- D:\Tesis\Modelo 3D\CAD\Electronicos\MC15A_V5\MC15A_V5_1779569544.214\MC15A_V5_1779569544.214\eMachineShop.20.284.ipt
- D:\Tesis\Modelo 3D\CAD\Electronicos\MC15A_V5\MC15A_V5_1779569544.214\MC15A_V5_1779569544.214\eMachineShop.20.285.ipt
- D:\Tesis\Modelo 3D\CAD\Electronicos\MC15A_V5\MC15A_V5_1779569544.214\MC15A_V5_1779569544.214\eMachineShop.20.286.ipt
- D:\Tesis\Modelo 3D\CAD\Electronicos\MC15A_V5\MC15A_V5_1779569544.214\MC15A_V5_1779569544.214\eMachineShop.20.287.ipt
- D:\Tesis\Modelo 3D\CAD\Electronicos\MC15A_V5\MC15A_V5_1779569544.214\MC15A_V5_1779569544.214\eMachineShop.20.288.ipt
- D:\Tesis\Modelo 3D\CAD\Electronicos\MC15A_V5\MC15A_V5_1779569544.214\MC15A_V5_1779569544.214\eMachineShop.20.289.ipt
- D:\Tesis\Modelo 3D\CAD\Electronicos\MC15A_V5\MC15A_V5_1779569544.214\MC15A_V5_1779569544.214\eMachineShop.20.290.ipt
- D:\Tesis\Modelo 3D\CAD\Electronicos\MC15A_V5\MC15A_V5_1779569544.214\MC15A_V5_1779569544.214\eMachineShop.20.291.ipt
- D:\Tesis\Modelo 3D\CAD\Electronicos\MC15A_V5\MC15A_V5_1779569544.214\MC15A_V5_1779569544.214\eMachineShop.20.292.ipt
- D:\Tesis\Modelo 3D\CAD\Electronicos\MC15A_V5\MC15A_V5_1779569544.214\MC15A_V5_1779569544.214\eMachineShop.20.293.ipt
- D:\Tesis\Modelo 3D\CAD\Electronicos\MC15A_V5\MC15A_V5_1779569544.214\MC15A_V5_1779569544.214\eMachineShop.20.294.ipt
- D:\Tesis\Modelo 3D\CAD\Electronicos\MC15A_V5\MC15A_V5_1779569544.214\MC15A_V5_1779569544.214\eMachineShop.20.295.ipt
- D:\Tesis\Modelo 3D\CAD\Electronicos\MC15A_V5\MC15A_V5_1779569544.214\MC15A_V5_1779569544.214\eMachineShop.20.296.ipt
- D:\Tesis\Modelo 3D\CAD\Electronicos\MC15A_V5\MC15A_V5_1779569544.214\MC15A_V5_1779569544.214\eMachineShop.20.297.ipt
- D:\Tesis\Modelo 3D\CAD\Electronicos\MC15A_V5\MC15A_V5_1779569544.214\MC15A_V5_1779569544.214\eMachineShop.20.298.ipt
- D:\Tesis\Modelo 3D\CAD\Electronicos\MC15A_V5\MC15A_V5_1779569544.214\MC15A_V5_1779569544.214\eMachineShop.20.299.ipt
- D:\Tesis\Modelo 3D\CAD\Electronicos\MC15A_V5\MC15A_V5_1779569544.214\MC15A_V5_1779569544.214\eMachineShop.20.300.ipt
- D:\Tesis\Modelo 3D\CAD\Electronicos\MC15A_V5\MC15A_V5_1779569544.214\MC15A_V5_1779569544.214\eMachineShop.20.301.ipt
- D:\Tesis\Modelo 3D\CAD\Electronicos\MC15A_V5\MC15A_V5_1779569544.214\MC15A_V5_1779569544.214\eMachineShop.20.302.ipt
- D:\Tesis\Modelo 3D\CAD\Electronicos\MC15A_V5\MC15A_V5_1779569544.214\MC15A_V5_1779569544.214\eMachineShop.20.303.ipt
- D:\Tesis\Modelo 3D\CAD\Electronicos\MC15A_V5\MC15A_V5_1779569544.214\MC15A_V5_1779569544.214\eMachineShop.20.304.ipt
- D:\Tesis\Modelo 3D\CAD\Electronicos\MC15A_V5\MC15A_V5_1779569544.214\MC15A_V5_1779569544.214\eMachineShop.20.305.ipt
- D:\Tesis\Modelo 3D\CAD\Electronicos\MC15A_V5\MC15A_V5_1779569544.214\MC15A_V5_1779569544.214\eMachineShop.20.306.ipt
- D:\Tesis\Modelo 3D\CAD\Electronicos\MC15A_V5\MC15A_V5_1779569544.214\MC15A_V5_1779569544.214\eMachineShop.20.307.ipt
- D:\Tesis\Modelo 3D\CAD\Electronicos\MC15A_V5\MC15A_V5_1779569544.214\MC15A_V5_1779569544.214\eMachineShop.20.308.ipt
- D:\Tesis\Modelo 3D\CAD\Electronicos\MC15A_V5\MC15A_V5_1779569544.214\MC15A_V5_1779569544.214\eMachineShop.20.309.ipt
- D:\Tesis\Modelo 3D\CAD\Electronicos\MC15A_V5\MC15A_V5_1779569544.214\MC15A_V5_1779569544.214\eMachineShop.20.310.ipt
- D:\Tesis\Modelo 3D\CAD\Electronicos\MC15A_V5\MC15A_V5_1779569544.214\MC15A_V5_1779569544.214\eMachineShop.20.311.ipt
- D:\Tesis\Modelo 3D\CAD\Electronicos\MC15A_V5\MC15A_V5_1779569544.214\MC15A_V5_1779569544.214\eMachineShop.20.312.ipt
- D:\Tesis\Modelo 3D\CAD\Electronicos\MC15A_V5\MC15A_V5_1779569544.214\MC15A_V5_1779569544.214\eMachineShop.20.313.ipt
- D:\Tesis\Modelo 3D\CAD\Electronicos\MC15A_V5\MC15A_V5_1779569544.214\MC15A_V5_1779569544.214\eMachineShop.20.314.ipt